# Autodesk Inventor assembly: SDS MK4i Swerve Module NEOS
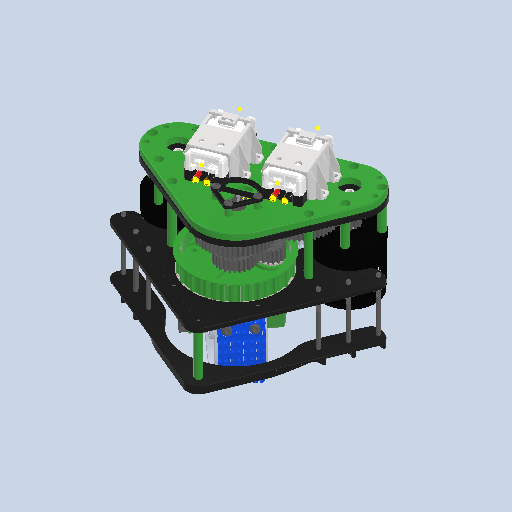
[picture p0: Inventor's stored thumbnail of the model, 512x512]
Saved by Autodesk Inventor 2023 (Build 270158000, 158)
## iProperties
Created: 2023-03-28
Part Number: SDS MK4i Swerve Module NEOS
Document SubType Name: Assembly
Designer: jackc
Author: jackc
## Documents named in this file (8)
- G:\.shortcut-targets-by-id\1MkDWIt6nIPqRnJSGLfoCUaNz0aFopGUn\1939_Arnold\2_Design\2023-2024\Parts\Swerve\SDS MK4i Swerve Module NEOS.iam
- G:\.shortcut-targets-by-id\1MkDWIt6nIPqRnJSGLfoCUaNz0aFopGUn\1939_Arnold\2_Design\2023-2024\Parts\Swerve\NEO Drive Gear.iam
- G:\.shortcut-targets-by-id\1MkDWIt6nIPqRnJSGLfoCUaNz0aFopGUn\1939_Arnold\2_Design\2023-2024\Parts\Swerve\NEO Turn Gear.iam
- G:\.shortcut-targets-by-id\1MkDWIt6nIPqRnJSGLfoCUaNz0aFopGUn\1939_Arnold\2_Design\2023-2024\Parts\Swerve\SDS MK4i Swerve Module, unpopulated.iam
- G:\.shortcut-targets-by-id\1MkDWIt6nIPqRnJSGLfoCUaNz0aFopGUn\1939_Arnold\2_Design\2023-2024\Parts\Motors\REV-21-1650 (NEO).ipt
- G:\.shortcut-targets-by-id\1MkDWIt6nIPqRnJSGLfoCUaNz0aFopGUn\1939_Arnold\2_Design\2023-2024\Parts\Printed Parts\Module_SPM_Mount.ipt
- G:\.shortcut-targets-by-id\1MkDWIt6nIPqRnJSGLfoCUaNz0aFopGUn\1939_Arnold\2_Design\2023-2024\Parts\Electronics\REV-11-2158-Spark-MAX.ipt
- G:\.shortcut-targets-by-id\1MkDWIt6nIPqRnJSGLfoCUaNz0aFopGUn\1939_Arnold\2_Design\2023-2024\Parts\Electronics\REV-21-2151_SPM_Mount.ipt
## Components (10 placed, 7 different names)
1. NEO Drive Gear:1 [sub-assembly]
2. NEO Turn Gear:1 [sub-assembly]
3. SDS MK4i Swerve Module, unpopulated:1 [sub-assembly] — Mate:13, Mate:14, Mate:15, Mate:16, Mate:17, Mate:18
4. REV-21-1650 (NEO):1 — Mate:13, Mate:14, Mate:15
5. REV-21-1650 (NEO):2 — Mate:16, Mate:17, Mate:18
6. Module_SPM_Mount:1
7. REV-11-2158-Spark-MAX:1
8. REV-11-2158-Spark-MAX:2
9. REV-21-2151_SPM_Mount:1
10. REV-21-2151_SPM_Mount:2
## Relationships (24: Mate 18, Angle 4, Flush 1, Tangent 1)
- [Mate]: SDS MK4i Swerve Module, unpopulated:1 ↔ Module_SPM_Mount:1
- [Mate]: SDS MK4i Swerve Module, unpopulated:1 ↔ Module_SPM_Mount:1
- [Mate]: SDS MK4i Swerve Module, unpopulated:1 ↔ Module_SPM_Mount:1
- [Mate]: SDS MK4i Swerve Module, unpopulated:1 ↔ Module_SPM_Mount:1
- [Angle] (180 deg): SDS MK4i Swerve Module, unpopulated:1 ↔ Module_SPM_Mount:1
- [Mate]: SDS MK4i Swerve Module, unpopulated:1 ↔ Module_SPM_Mount:1
- [Mate]: Module_SPM_Mount:1 ↔ REV-11-2158-Spark-MAX:2
- [Mate]: Module_SPM_Mount:1 ↔ REV-11-2158-Spark-MAX:1
- [Flush] (5.08 mm): Module_SPM_Mount:1 ↔ REV-11-2158-Spark-MAX:1
- [Mate]: REV-11-2158-Spark-MAX:2 ↔ REV-21-2151_SPM_Mount:1
- [Angle] (0 deg): REV-11-2158-Spark-MAX:2 ↔ REV-21-2151_SPM_Mount:1
- [Mate]: Module_SPM_Mount:1 ↔ REV-21-2151_SPM_Mount:1
- [Mate]: REV-11-2158-Spark-MAX:1 ↔ REV-21-2151_SPM_Mount:2
- [Angle] (0 deg): REV-11-2158-Spark-MAX:1 ↔ REV-21-2151_SPM_Mount:2
- [Mate]: Module_SPM_Mount:1 ↔ REV-21-2151_SPM_Mount:2
- [Tangent] (4.445 mm): SDS MK4i Swerve Module, unpopulated:1 ↔ REV-21-2151_SPM_Mount:2
- [Mate]: Module_SPM_Mount:1 ↔ REV-21-2151_SPM_Mount:1
- [Angle] (90 deg): Module_SPM_Mount:1 ↔ REV-11-2158-Spark-MAX:2
- Mate:13: SDS MK4i Swerve Module, unpopulated:1 ↔ REV-21-1650 (NEO):1
- Mate:14: SDS MK4i Swerve Module, unpopulated:1 ↔ REV-21-1650 (NEO):1
- Mate:15: SDS MK4i Swerve Module, unpopulated:1 ↔ REV-21-1650 (NEO):1
- Mate:16: SDS MK4i Swerve Module, unpopulated:1 ↔ REV-21-1650 (NEO):2
- Mate:17: SDS MK4i Swerve Module, unpopulated:1 ↔ REV-21-1650 (NEO):2
- Mate:18: SDS MK4i Swerve Module, unpopulated:1 ↔ REV-21-1650 (NEO):2
